# Autodesk Inventor assembly: WheelIntake4.0
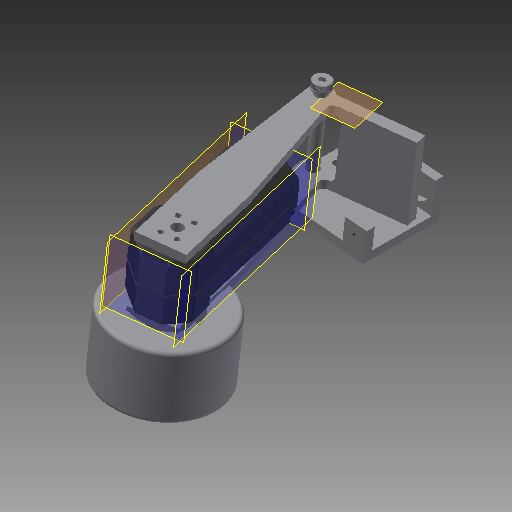
[picture p0: Inventor's stored thumbnail of the model, 512x512]
Saved by Autodesk Inventor 2017 SP1 (Build 210196100, 196)
## iProperties
Created: 2017-12-13
Part Number: WheelIntake4.0
Document SubType Name: Assembly
Designer: User
Author: User
## Documents named in this file (6)
- C:\robotics\CAD\2017-18_CAD\WheelIntake5.0.iam
- C:\robotics\CAD\COTSParts\Rev\REV-41-1300.ipt
- C:\robotics\CAD\COTSParts\Fasteners\97345A171_TYPE 316 STAINLESS STEEL SHOULDER SCREW.ipt
- C:\robotics\CAD\COTSParts\Wheels\2.5inFoamWheel250TMD.ipt
- C:\robotics\CAD\2017-18_CAD\WheelIntake5.0Base.ipt
- C:\robotics\CAD\2017-18_CAD\WheelIntake5.0Mount.ipt
## Components (5 placed, 5 different names)
1. REV-41-1300:1 — Insert:2, Insert:3
2. 97345A171_TYPE 316 STAINLESS STEEL SHOULDER SCREW:1 — Insert:1, Insert:8
3. 2.5inFoamWheel250TMD:1 — Insert:7
4. WheelIntake5.0Base:1 — Insert:8
5. WheelIntake5.0Mount:1 — Insert:1, Insert:2, Insert:3, Insert:7
## Relationships (5: Insert 5)
- Insert:1: 97345A171_TYPE 316 STAINLESS STEEL SHOULDER SCREW:1 ↔ WheelIntake5.0Mount:1
- Insert:2: REV-41-1300:1 ↔ WheelIntake5.0Mount:1
- Insert:3: REV-41-1300:1 ↔ WheelIntake5.0Mount:1
- Insert:7: 2.5inFoamWheel250TMD:1 ↔ WheelIntake5.0Mount:1
- Insert:8: 97345A171_TYPE 316 STAINLESS STEEL SHOULDER SCREW:1 ↔ WheelIntake5.0Base:1
